# Autodesk Inventor assembly: CLB_068_GrooveBearingSlider
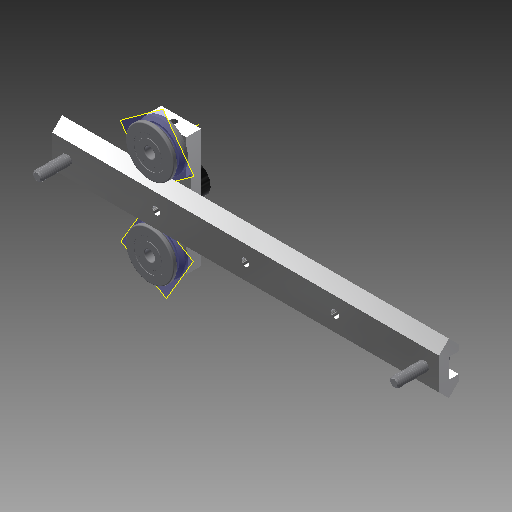
[picture p0: Inventor's stored thumbnail of the model, 512x512]
Saved by Autodesk Inventor 2018.3 (Build 223284000, 284)
## iProperties
Created: 2020-02-15
Part Number: CLB_068_GrooveBearingSlider
Document SubType Name: Assembly
Designer: 22jungchan
Author: 22jungchan
## Documents named in this file (6)
- C:\Users\myerpaul\Documents\GrabCAD\Infinite Recharge 2020\Build season\CLB_068_GrooveBearingSlider.iam
- C:\Users\myerpaul\Documents\GrabCAD\Infinite Recharge 2020\Build season\CLB_069_GrooveBearingSliderPath.ipt
- C:\Users\myerpaul\Documents\GrabCAD\Infinite Recharge 2020\Build season\CLB_070_RollerBracket.ipt
- C:\Users\myerpaul\Documents\GrabCAD\Infinite Recharge 2020\Build season\CLB_067_W2RXBearing.ipt
- C:\Users\myerpaul\Documents\GrabCAD\Infinite Recharge 2020\Build season\CLB_071_CapScrew.ipt
- C:\Users\myerpaul\Documents\GrabCAD\Infinite Recharge 2020\Build season\CLB_050_ScissorSliderSpacer.ipt
## Components (7 placed, 5 different names)
1. CLB_069_GrooveBearingSliderPath:1 — Mate:6, Mate:8, Insert:9, Insert:10
2. CLB_070_RollerBracket:1 — Mate:3, Insert:6, Insert:8, Mate:7, Mate:8
3. CLB_067_W2RXBearing:1 — Flush:1, Mate:7
4. CLB_067_W2RXBearing:2 — Insert:8, Mate:6, Flush:1
5. CLB_071_CapScrew:1 — Insert:9
6. CLB_050_ScissorSliderSpacer:1 — Mate:3, Insert:6
7. CLB_071_CapScrew:2 — Insert:10
## Relationships (9: Mate 4, Insert 4, Flush 1)
- Mate:3: CLB_070_RollerBracket:1 ↔ CLB_050_ScissorSliderSpacer:1
- Insert:6: CLB_070_RollerBracket:1 ↔ CLB_050_ScissorSliderSpacer:1
- Insert:8 (1.5875 mm): CLB_070_RollerBracket:1 ↔ CLB_067_W2RXBearing:2
- Flush:1: CLB_067_W2RXBearing:1 ↔ CLB_067_W2RXBearing:2
- Mate:6: CLB_069_GrooveBearingSliderPath:1 ↔ CLB_067_W2RXBearing:2
- Mate:7: CLB_070_RollerBracket:1 ↔ CLB_067_W2RXBearing:1
- Mate:8: CLB_069_GrooveBearingSliderPath:1 ↔ CLB_070_RollerBracket:1
- Insert:9: CLB_069_GrooveBearingSliderPath:1 ↔ CLB_071_CapScrew:1
- Insert:10: CLB_069_GrooveBearingSliderPath:1 ↔ CLB_071_CapScrew:2
